# Autodesk Inventor assembly: Тиски_сборка
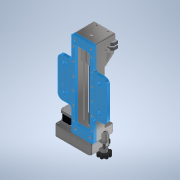
[picture p0: Inventor's stored thumbnail of the model, 180x180]
Saved by Autodesk Inventor 2021 (Build 250183000, 183)
## iProperties
Created: 2020-12-08
Part Number: Тиски_сборка
Document SubType Name: Assembly
Designer: User
Mass: 8164.5 g
Surface Area: 3956.63 cm^2
Volume: 1309.47 cm^3
Density: 6.23498 g/cm^3
Author: User
## Documents named in this file (21)
- F:\Vise\Модели\Тиски\Тиски_сборка.iam
- F:\Vise\Модели\Тиски\Основание.ipt
- F:\Vise\Модели\Тиски\Упор 1.ipt
- F:\Vise\Модели\Тиски\Направляющая.ipt
- F:\Vise\Модели\Тиски\Упор 2.ipt
- F:\Vise\Модели\Тиски\Вал1.ipt
- F:\Vise\Модели\Тиски\Тиски\Мастер проектирования\Подшипник1.iam
- F:\Vise\Модели\Тиски\Фланец_1.ipt
- C:\Users\User\Documents\Inventor\Content Center Files\R2020\ru-RU\DIN 916\DIN 916 - M4  x  10.ipt
- F:\Vise\Модели\Тиски\Каретка.ipt
- F:\Vise\Модели\Тиски\Губка.ipt
- F:\Vise\Модели\Тиски\Тиски_сборка\Мастер проектирования\Болтовое соединение1.iam
- F:\Vise\Модели\Тиски\Тиски_сборка\Мастер проектирования\Болтовое соединение2.iam
- F:\Vise\Модели\Тиски\Тиски_сборка\Мастер проектирования\Болтовое соединение3.iam
- F:\Vise\Модели\Тиски\Тиски_сборка\Мастер проектирования\Болтовое соединение4.iam
- F:\Vise\Модели\Тиски\Ручной привод.iam
- F:\Vise\Модели\Тиски\Тиски_сборка\Мастер проектирования\Болтовое соединение5.iam
- F:\Vise\Модели\Тиски\Колпачок.ipt
- F:\Vise\Модели\Тиски\Привод.iam
- F:\Vise\Модели\Тиски\Тиски_сборка\Мастер проектирования\Болтовое соединение6.iam
- F:\Vise\Модели\Тиски\Ручка.ipt
## Components (25 placed, 15 different names)
1. Основание:1 — Заподлицо:1, Заподлицо:2, Совмещение:1, Жесткий:1, Жесткий:3, Совмещение:3, Совмещение:4, Совмещение:5, Совмещение:6
2. Упор 1:1 — Жесткий:1, Жесткий:2, Жесткий:4, Жесткий:10, Совмещение:19
3. Направляющая:1 — Жесткий:2, Заподлицо:3, Совмещение:20
4. Упор 2:1 — Жесткий:3, Жесткий:5, Совмещение:27, Совмещение:28
5. Вал:1 — С поворотом:1, Жесткий:6, Совмещение:2, Жесткий:11, С поворотом:2
6. Подшипник:1 [sub-assembly] — Жесткий:4
7. Подшипник:2 [sub-assembly] — Жесткий:5, С поворотом:1
8. Фланец_1:1 — Жесткий:6, Жесткий:7, Жесткий:8
9. DIN 916 M4  x  10:1 — Жесткий:7
10. DIN 916 M4  x  10:2 — Жесткий:8
11. Каретка:1 — Совмещение:2, Заподлицо:3, Жесткий:9
12. Губка:1 — Жесткий:9, Совмещение:9, Совмещение:10, Совмещение:29
13. Губка:2 — Жесткий:10, Совмещение:7, Совмещение:8, Совмещение:16
14. Болтовое соединение:1 [sub-assembly] — Совмещение:3, Совмещение:4, Совмещение:20
15. Болтовое соединение:2 [sub-assembly] — Совмещение:5, Совмещение:6, Совмещение:19
16. Болтовое соединение:3 [sub-assembly] — Совмещение:7, Совмещение:8, Совмещение:16
17. Болтовое соединение:4 [sub-assembly] — Совмещение:9, Совмещение:10, Совмещение:29
18. Ручной привод:1 [sub-assembly] — Жесткий:11, Совмещение:11, Совмещение:12
19. Болтовое соединение:5 [sub-assembly] — Совмещение:11, Совмещение:12, Заподлицо:4, Жесткий:12
20. Колпачок:1 — Заподлицо:4
21. Колпачок:2 — Жесткий:12
22. Привод:1 [sub-assembly] — С поворотом:2, Совмещение:14, Совмещение:15, Совмещение:27
23. Болтовое соединение:6 [sub-assembly] — Совмещение:14, Совмещение:15, Совмещение:21, Совмещение:22, Совмещение:23, Совмещение:24, Совмещение:25, Совмещение:26, Совмещение:28
24. Ручка:1 — Совмещение:24, Совмещение:25, Совмещение:26
25. Ручка:2 — Совмещение:21, Совмещение:22, Совмещение:23
## Relationships (44: Mate 26, WeldJoint 12, Flush 4, RevoluteJoint 2)
- Заподлицо:1 [Flush]: Основание:1
- Заподлицо:2 [Flush]: Основание:1
- Совмещение:1 [Mate]: Основание:1
- Жесткий:1 [WeldJoint]: Основание:1 ↔ Упор 1:1
- Жесткий:2 [WeldJoint]: Упор 1:1 ↔ Направляющая:1
- Жесткий:3 [WeldJoint]: Основание:1 ↔ Упор 2:1
- Жесткий:4 [WeldJoint]: Упор 1:1 ↔ Подшипник:1
- Жесткий:5 [WeldJoint]: Упор 2:1 ↔ Подшипник:2
- С поворотом:1 [RevoluteJoint]: Вал:1 ↔ Подшипник:2
- Жесткий:6 [WeldJoint] (-16 mm): Вал:1 ↔ Фланец_1:1
- Жесткий:7 [WeldJoint] (-1 mm): Фланец_1:1 ↔ DIN 916 M4  x  10:1
- Жесткий:8 [WeldJoint] (-1 mm): Фланец_1:1 ↔ DIN 916 M4  x  10:2
- Совмещение:2 [Mate]: Вал:1 ↔ Каретка:1
- Заподлицо:3 [Flush]: Направляющая:1 ↔ Каретка:1
- Жесткий:9 [WeldJoint]: Каретка:1 ↔ Губка:1
- Жесткий:10 [WeldJoint]: Упор 1:1 ↔ Губка:2
- Совмещение:3 [Mate]: Основание:1 ↔ Болтовое соединение:1
- Совмещение:4 [Mate]: Основание:1 ↔ Болтовое соединение:1
- Совмещение:5 [Mate]: Основание:1 ↔ Болтовое соединение:2
- Совмещение:6 [Mate]: Основание:1 ↔ Болтовое соединение:2
- Совмещение:7 [Mate]: Губка:2 ↔ Болтовое соединение:3
- Совмещение:8 [Mate]: Губка:2 ↔ Болтовое соединение:3
- Совмещение:9 [Mate]: Губка:1 ↔ Болтовое соединение:4
- Совмещение:10 [Mate]: Губка:1 ↔ Болтовое соединение:4
- Жесткий:11 [WeldJoint]: Вал:1 ↔ Ручной привод:1
- Совмещение:11 [Mate]: Ручной привод:1 ↔ Болтовое соединение:5
- Совмещение:12 [Mate]: Ручной привод:1 ↔ Болтовое соединение:5
- Заподлицо:4 [Flush]: Болтовое соединение:5 ↔ Колпачок:1
- Жесткий:12 [WeldJoint]: Болтовое соединение:5 ↔ Колпачок:2
- С поворотом:2 [RevoluteJoint] (-16 mm): Вал:1 ↔ Привод:1
- Совмещение:14 [Mate]: Привод:1 ↔ Болтовое соединение:6
- Совмещение:15 [Mate]: Привод:1 ↔ Болтовое соединение:6
- Совмещение:16 [Mate]: Губка:2 ↔ Болтовое соединение:3
- Совмещение:19 [Mate]: Упор 1:1 ↔ Болтовое соединение:2
- Совмещение:20 [Mate]: Направляющая:1 ↔ Болтовое соединение:1
- Совмещение:21 [Mate]: Болтовое соединение:6 ↔ Ручка:2
- Совмещение:22 [Mate]: Болтовое соединение:6 ↔ Ручка:2
- Совмещение:23 [Mate]: Болтовое соединение:6 ↔ Ручка:2
- Совмещение:24 [Mate]: Болтовое соединение:6 ↔ Ручка:1
- Совмещение:25 [Mate]: Болтовое соединение:6 ↔ Ручка:1
- Совмещение:26 [Mate]: Болтовое соединение:6 ↔ Ручка:1
- Совмещение:27 [Mate]: Упор 2:1 ↔ Привод:1
- Совмещение:28 [Mate]: Упор 2:1 ↔ Болтовое соединение:6
- Совмещение:29 [Mate]: Губка:1 ↔ Болтовое соединение:4
